# Autodesk Inventor assembly: ToolLockAssy
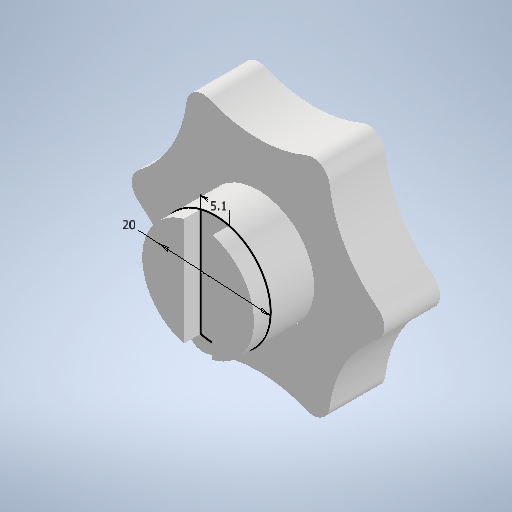
[picture p0: Inventor's stored thumbnail of the model, 512x512]
Saved by Autodesk Inventor 2025.3 (Build 293356030, 356C)
## iProperties
Created: 2025-10-10
Part Number: ToolLockAssy
Document SubType Name: Assembly
Designer: tvoko
Author: tvoko
## Documents named in this file (3)
- C:\Users\tvoko\Github\DIY-Coil-Winder\CAD\ToolLockAssy.iam
- C:\Users\tvoko\Github\DIY-Coil-Winder\CAD\Tool-lock-Slot.ipt
- C:\Users\tvoko\Github\DIY-Coil-Winder\CAD\Tool-Lock-Knob.ipt
## Components (2 placed, 2 different names)
1. Tool-lock-Slot:1 — Mate:1
2. Tool-Lock-Knob:1 — Mate:1
## Relationships (1: Mate 1)
- Mate:1: Tool-lock-Slot:1 ↔ Tool-Lock-Knob:1
